# Autodesk Inventor assembly: Alabes y pines
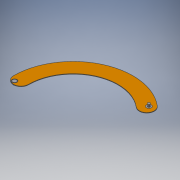
[picture p0: Inventor's stored thumbnail of the model, 180x180]
Saved by Autodesk Inventor 2019 (Build 230136000, 136)
## iProperties
Created: 2020-08-28
Part Number: Alabes y pines
Document SubType Name: Assembly
Designer: Hugo Albarracin
Author: Hugo Albarracin
## Documents named in this file (3)
- C:\Users\Hugo Albarracin\OneDrive - Escuela Superior Politécnica del Litoral\U - UPM ELECTROMECANICA\14. TFM\iris_mecanico\Alabes y pines.iam
- C:\Users\Hugo Albarracin\OneDrive - Escuela Superior Politécnica del Litoral\U - UPM ELECTROMECANICA\14. TFM\iris_mecanico\Alabes.ipt
- C:\Users\Hugo Albarracin\OneDrive - Escuela Superior Politécnica del Litoral\U - UPM ELECTROMECANICA\14. TFM\iris_mecanico\Alabe_pivote.ipt
## Components (3 placed, 2 different names)
1. Alabes:1 — Mate:1, Flush:1, Mate:2, Flush:2
2. Alabe_pivote:1 — Mate:2, Flush:2
3. Alabe_pivote:2 — Mate:1, Flush:1
## Relationships (4: Mate 2, Flush 2)
- Mate:1: Alabes:1 ↔ Alabe_pivote:2
- Flush:1: Alabes:1 ↔ Alabe_pivote:2
- Mate:2: Alabes:1 ↔ Alabe_pivote:1
- Flush:2: Alabes:1 ↔ Alabe_pivote:1
